# Autodesk Inventor assembly: MainMount
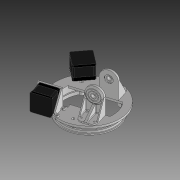
[picture p0: Inventor's stored thumbnail of the model, 180x180]
Saved by Autodesk Inventor 2020 (Build 240168000, 168)
## iProperties
Created: 2020-09-16
Part Number: MainMount
Document SubType Name: Assembly
Designer: DDeGo
Author: DDeGo
## Documents named in this file (7)
- C:\Users\DDeGo\Documents\Drew\Projects\Nerf Aim Assist\Cad\MainMount.iam
- C:\Users\DDeGo\Documents\Drew\Projects\Nerf Aim Assist\Cad\BearingBracket.ipt
- C:\Users\DDeGo\Documents\Drew\Projects\Nerf Aim Assist\Cad\SwivelMount.ipt
- C:\Users\DDeGo\Documents\Drew\Projects\Nerf Aim Assist\Cad\608zz.ipt
- C:\Users\DDeGo\Documents\Drew\Projects\Nerf Aim Assist\Cad\Nema 17.ipt
- C:\Users\DDeGo\Documents\Drew\Projects\Nerf Aim Assist\Cad\PitchMotorBracket.ipt
- C:\Users\DDeGo\Documents\Drew\Projects\Nerf Aim Assist\Cad\SwivelMountClamp.ipt
## Components (9 placed, 6 different names)
1. BearingBracket:1 — Mate:3, Mate:6, Mate:9, Mate:10, Mate:12
2. SwivelMount:1 — Mate:3, Mate:4, Mate:7, Mate:8, Mate:9, Mate:10, Mate:13, Mate:14, Mate:15, Mate:16, Mate:17, Mate:18, Mate:22, Mate:23, Mate:24
3. BearingBracket:2 — Mate:4, Mate:5, Mate:7, Mate:8, Mate:11
4. 608zz:1 — Mate:5, Mate:11
5. 608zz:2 — Mate:6, Mate:12
6. Nema 17:1 — Mate:13, Mate:14, Mate:15
7. Nema 17:2 — Mate:19, Mate:20, Mate:21
8. PitchMotorBracket:1 — Mate:16, Mate:17, Mate:18, Mate:19, Mate:20, Mate:21
9. SwivelMountClamp:1 — Mate:22, Mate:23, Mate:24
## Relationships (22: Mate 22)
- Mate:3: BearingBracket:1 ↔ SwivelMount:1
- Mate:4: SwivelMount:1 ↔ BearingBracket:2
- Mate:5: BearingBracket:2 ↔ 608zz:1
- Mate:6: BearingBracket:1 ↔ 608zz:2
- Mate:7: SwivelMount:1 ↔ BearingBracket:2
- Mate:8: SwivelMount:1 ↔ BearingBracket:2
- Mate:9: BearingBracket:1 ↔ SwivelMount:1
- Mate:10: BearingBracket:1 ↔ SwivelMount:1
- Mate:11: BearingBracket:2 ↔ 608zz:1
- Mate:12: BearingBracket:1 ↔ 608zz:2
- Mate:13: SwivelMount:1 ↔ Nema 17:1
- Mate:14: SwivelMount:1 ↔ Nema 17:1
- Mate:15: SwivelMount:1 ↔ Nema 17:1
- Mate:16: SwivelMount:1 ↔ PitchMotorBracket:1
- Mate:17: SwivelMount:1 ↔ PitchMotorBracket:1
- Mate:18: SwivelMount:1 ↔ PitchMotorBracket:1
- Mate:19: Nema 17:2 ↔ PitchMotorBracket:1
- Mate:20: Nema 17:2 ↔ PitchMotorBracket:1
- Mate:21: Nema 17:2 ↔ PitchMotorBracket:1
- Mate:22: SwivelMount:1 ↔ SwivelMountClamp:1
- Mate:23: SwivelMount:1 ↔ SwivelMountClamp:1
- Mate:24 (12.7 mm): SwivelMount:1 ↔ SwivelMountClamp:1
